# Autodesk Inventor assembly: front-right-holder
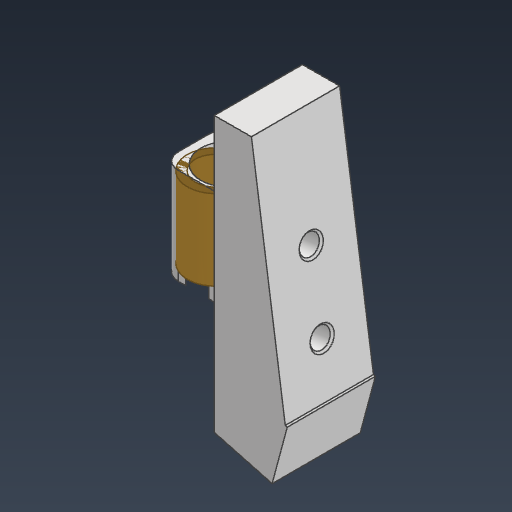
[picture p0: Inventor's stored thumbnail of the model, 512x512]
Saved by Autodesk Inventor 2023 (Build 270158000, 158)
## iProperties
Created: 2025-03-31
Part Number: front-right-holder
Document SubType Name: Assembly
Designer: szymo
Author: szymo
## Documents named in this file (3)
- D:\tech\robotyka\robots\evangelion\inventor-project\front-right-holder.iam
- D:\tech\robotyka\robots\evangelion\inventor-project\lozysko sf-1.ipt
- D:\tech\robotyka\robots\evangelion\inventor-project\front-hold-rght.ipt
## Components (2 placed, 2 different names)
1. front-hold-rght:1 — Mate:1, Mate:2
2. lozysko sf-1:1 — Mate:1, Mate:2
## Relationships (2: Mate 2)
- Mate:1: front-hold-rght:1 ↔ lozysko sf-1:1
- Mate:2: front-hold-rght:1 ↔ lozysko sf-1:1
